# Autodesk Inventor assembly: Mold Design1
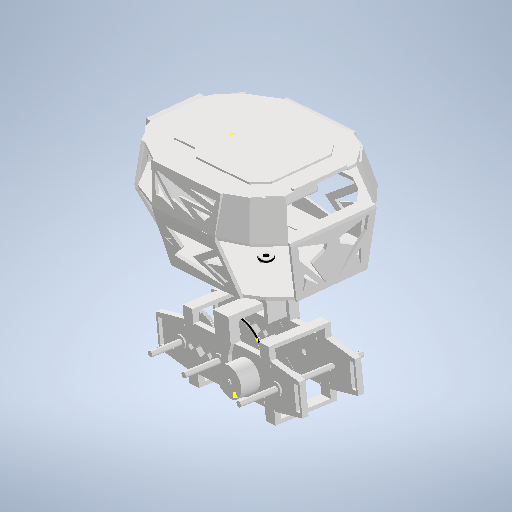
[picture p0: Inventor's stored thumbnail of the model, 512x512]
Saved by Autodesk Inventor 2025.2 (Build 292293000, 293)
## iProperties
Created: 2025-04-15
Part Number: Mold Design1
Document SubType Name: Assembly
Designer: ziyuz
Author: ziyuz
## Documents named in this file (17)
- F:\autoeskinvetersave\lanche\Mold Design1.iam
- F:\autoeskinvetersave\lanche\Part1EDDV4.ipt
- F:\autoeskinvetersave\lanche\Part2EDD.ipt
- F:\autoeskinvetersave\lanche\Part3EDD.ipt
- F:\autoeskinvetersave\lanche\Part4EDD.ipt
- F:\autoeskinvetersave\lanche\Part6.ipt
- F:\autoeskinvetersave\lanchetop\Connecting pt.1.ipt
- F:\autoeskinvetersave\lanchetop\Connecting pt.2.ipt
- F:\autoeskinvetersave\lanchetop\Side w motor.ipt
- F:\autoeskinvetersave\lanchetop\SideV1.ipt
- F:\autoeskinvetersave\Part3.ipt
- F:\autoeskinvetersave\Part6.ipt
- F:\autoeskinvetersave\Part5.ipt
- F:\autoeskinvetersave\Part9.ipt
- F:\autoeskinvetersave\Part8.ipt
- F:\autoeskinvetersave\Part7.ipt
- F:\autoeskinvetersave\Part4.ipt
## Components (29 placed, 15 different names)
1. Part1EDDV4:1 — Rigid:1, Rotational:1, Rotational:2, Rotational:3, Mate:1, Mate:2, Mate:3
2. Part2EDD:1 — Rigid:1
3. Part3EDD:1 — Rotational:2
4. Part3EDD:2 — Rotational:3
5. Part4EDD:1 — Rotational:1, Mate:8, Mate:9
6. Part6:1 — Mate:1, Mate:2, Mate:3
7. Connecting pt.1:1 — Mate:8, Mate:9, Rigid:2
8. Connecting pt.2:1 — Mate:6, Mate:7, Flush:2, Rigid:2
9. Side w motor:1 — Mate:6, Mate:7, Flush:2, Mate:10, Mate:15, Flush:5, Mate:16, Flush:6, Mate:17, Rotational:4, Mate:21, Rotational:14, Rotational:15, Rotational:16
10. Part3:1 — Mate:10, Mate:18, Mate:19, Flush:7
11. Part3:2
12. Part3:3 — Mate:15, Flush:5, Mate:20, Mate:21
13. Part3:4 — Mate:16, Flush:6, Mate:17
14. Part6:2 — Rotational:4, Rotational:5
15. Part5:1 — Rotational:6, Rotational:9
16. Part5:2 — Rotational:7, Rotational:10
17. Part5:3 — Rotational:8
18. Part9:1 — Rotational:9
19. Part8:1
20. Part8:2 — Rotational:5
21. Part7:1 — Rotational:10
22. SideV1:1 — Mate:18, Mate:19, Flush:7, Mate:20, Rotational:6, Rotational:7, Rotational:8, Rotational:11, Rotational:12, Rotational:13
23. Part4:1
24. Part4:2 — Rotational:12
25. Part4:3 — Rotational:13
26. Part4:4 — Rotational:14
27. Part4:5 — Rotational:16
28. Part4:6 — Rotational:15
29. Part4:7 — Rotational:11
## Relationships (37: RevoluteJoint 16, Mate 15, Flush 4, WeldJoint 2)
- Rigid:1 [WeldJoint] (12.5 mm): Part1EDDV4:1 ↔ Part2EDD:1
- Rotational:1 [RevoluteJoint] (-0.5 mm): Part1EDDV4:1 ↔ Part4EDD:1
- Rotational:2 [RevoluteJoint]: Part1EDDV4:1 ↔ Part3EDD:1
- Rotational:3 [RevoluteJoint]: Part1EDDV4:1 ↔ Part3EDD:2
- Mate:1: Part1EDDV4:1 ↔ Part6:1
- Mate:2: Part1EDDV4:1 ↔ Part6:1
- Mate:3: Part1EDDV4:1 ↔ Part6:1
- Mate:6: Connecting pt.2:1 ↔ Side w motor:1
- Mate:7: Connecting pt.2:1 ↔ Side w motor:1
- Flush:2: Connecting pt.2:1 ↔ Side w motor:1
- Mate:8: Part4EDD:1 ↔ Connecting pt.1:1
- Mate:9: Part4EDD:1 ↔ Connecting pt.1:1
- Rigid:2 [WeldJoint]: Connecting pt.1:1 ↔ Connecting pt.2:1
- Mate:10: Side w motor:1 ↔ Part3:1
- Mate:15: Side w motor:1 ↔ Part3:3
- Flush:5: Side w motor:1 ↔ Part3:3
- Mate:16: Side w motor:1 ↔ Part3:4
- Flush:6: Side w motor:1 ↔ Part3:4
- Mate:17: Side w motor:1 ↔ Part3:4
- Rotational:4 [RevoluteJoint] (4 mm): Side w motor:1 ↔ Part6:2
- Rotational:5 [RevoluteJoint] (-3.5 mm): Part6:2 ↔ Part8:2
- Mate:18: Part3:1 ↔ SideV1:1
- Mate:19: Part3:1 ↔ SideV1:1
- Flush:7: Part3:1 ↔ SideV1:1
- Mate:20: Part3:3 ↔ SideV1:1
- Mate:21: Side w motor:1 ↔ Part3:3
- Rotational:6 [RevoluteJoint] (-25 mm): Part5:1 ↔ SideV1:1
- Rotational:7 [RevoluteJoint] (-29 mm): Part5:2 ↔ SideV1:1
- Rotational:8 [RevoluteJoint] (-23 mm): Part5:3 ↔ SideV1:1
- Rotational:9 [RevoluteJoint] (51.25 mm): Part5:1 ↔ Part9:1
- Rotational:10 [RevoluteJoint] (55 mm): Part5:2 ↔ Part7:1
- Rotational:11 [RevoluteJoint]: SideV1:1 ↔ Part4:7
- Rotational:12 [RevoluteJoint]: SideV1:1 ↔ Part4:2
- Rotational:13 [RevoluteJoint]: SideV1:1 ↔ Part4:3
- Rotational:14 [RevoluteJoint]: Side w motor:1 ↔ Part4:4
- Rotational:15 [RevoluteJoint]: Side w motor:1 ↔ Part4:6
- Rotational:16 [RevoluteJoint]: Side w motor:1 ↔ Part4:5
